# Autodesk Inventor assembly: assembly
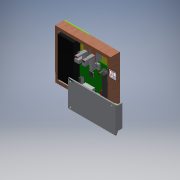
[picture p0: Inventor's stored thumbnail of the model, 180x180]
Saved by Autodesk Inventor 2017 (Build 210142000, 142)
## iProperties
Created: 2016-11-05
Part Number: assembly
Document SubType Name: Assembly
Designer: radrajith
Author: radrajith
## Documents named in this file (7)
- C:\Users\radra\Box Sync\Senior Fall 2016\ESE 323\autocad\assembly.iam
- C:\Users\radra\Box Sync\Senior Fall 2016\ESE 323\autocad\case_bottom.ipt
- C:\Users\radra\Box Sync\Senior Fall 2016\ESE 323\autocad\lab 04.ipt
- C:\Users\radra\Box Sync\Senior Fall 2016\ESE 323\autocad\battery.ipt
- C:\Users\radra\Box Sync\Senior Fall 2016\ESE 323\autocad\button_press.ipt
- C:\Users\radra\Documents\Inventor\Content Center Files\R2017\en-US\ANSI B18.2.4.2M\ANSI B18.2.4.2M - M3.5x0.6 - 6.ipt
- C:\Users\radra\Box Sync\Senior Fall 2016\ESE 323\autocad\lcd display.ipt
## Components (9 placed, 6 different names)
1. lab 04:1 — Insert:1, Insert:5, Mate:2, Mate:4, Mate:6, Mate:7, Mate:10
2. case_bottom:1 — Insert:1, Insert:5, Mate:1, Mate:3, Mate:5, Mate:8, Mate:9, Mate:11, Mate:12, Mate:13, Mate:14, Mate:15
3. battery:1 — Mate:13, Mate:14, Mate:15
4. button_press:1 — Mate:10, Mate:11, Mate:12
5. button_press:2 — Mate:7, Mate:8, Mate:9
6. ANSI B18.2.4.2M M3.5x0.6:1 — Mate:1, Mate:2
7. ANSI B18.2.4.2M M3.5x0.6:2 — Mate:3, Mate:4
8. ANSI B18.2.4.2M M3.5x0.6:3 — Mate:5, Mate:6
9. lcd display:1
## Relationships (17: Mate 15, Insert 2)
- Insert:1 (10 mm): lab 04:1 ↔ case_bottom:1
- Insert:5 (10 mm): lab 04:1 ↔ case_bottom:1
- Mate:1: case_bottom:1 ↔ ANSI B18.2.4.2M M3.5x0.6:1
- Mate:2: lab 04:1 ↔ ANSI B18.2.4.2M M3.5x0.6:1
- Mate:3: case_bottom:1 ↔ ANSI B18.2.4.2M M3.5x0.6:2
- Mate:4: lab 04:1 ↔ ANSI B18.2.4.2M M3.5x0.6:2
- Mate:5: case_bottom:1 ↔ ANSI B18.2.4.2M M3.5x0.6:3
- Mate:6: lab 04:1 ↔ ANSI B18.2.4.2M M3.5x0.6:3
- Mate:7: lab 04:1 ↔ button_press:2
- Mate:8: case_bottom:1 ↔ button_press:2
- Mate:9: case_bottom:1 ↔ button_press:2
- Mate:10: lab 04:1 ↔ button_press:1
- Mate:11: case_bottom:1 ↔ button_press:1
- Mate:12: case_bottom:1 ↔ button_press:1
- Mate:13: case_bottom:1 ↔ battery:1
- Mate:14: case_bottom:1 ↔ battery:1
- Mate:15: case_bottom:1 ↔ battery:1
